# Autodesk Inventor assembly: GE-12089
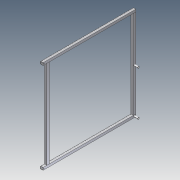
[picture p0: Inventor's stored thumbnail of the model, 180x180]
Saved by Autodesk Inventor 2012 (Build 160160000, 160)
## iProperties
Created: 2011-10-10
Part Number: GE-12089
Document SubType Name: Assembly
Designer: dfoster
Description: Corral Frame, Right
Title: Corral Frame, Right
Author: dfoster
## Documents named in this file (4)
- C:\Data Folder\FRC 2012 Field\Components\GE-12089.iam
- C:\Data Folder\FRC 2012 Field\Components\GE-12089-01.ipt
- C:\Data Folder\FRC 2012 Field\Components\GE-12089-02.ipt
- C:\Data Folder\FRC 2012 Field\Components\GE-12089-03.ipt
## Components (6 placed, 3 different names)
1. GE-12089-01:1 — Flush:1, Mate:1, Flush:2, Flush:3, Flush:5, Flush:6
2. GE-12089-01:2 — Mate:2, Flush:4, Flush:5
3. GE-12089-02:1 — Flush:1
4. GE-12089-02:2 — Mate:1, Flush:2, Flush:3, Mate:2, Flush:4
5. GE-12089-03:1 — Flush:6
6. GE-12089-03:2
## Relationships (13: Mate 7, Flush 6)
- Flush:1: GE-12089-01:1 ↔ GE-12089-02:1
- Mate:1: GE-12089-01:1 ↔ GE-12089-02:2
- Flush:2: GE-12089-01:1 ↔ GE-12089-02:2
- Flush:3 (50.8 mm): GE-12089-01:1 ↔ GE-12089-02:2
- Mate:2: GE-12089-01:2 ↔ GE-12089-02:2
- Flush:4: GE-12089-01:2 ↔ GE-12089-02:2
- Flush:5: GE-12089-01:1 ↔ GE-12089-01:2
- Flush:6: GE-12089-01:1 ↔ GE-12089-03:1
- [Mate] (-15.875 mm): GE-12089-01:1 ↔ GE-12089-03:1
- [Mate] (-15.875 mm): GE-12089-01:1 ↔ GE-12089-03:1
- [Mate]: GE-12089-02:1 ↔ GE-12089-03:2
- [Mate] (-15.875 mm): GE-12089-02:1 ↔ GE-12089-03:2
- [Mate] (-593.725 mm): GE-12089-01:1 ↔ GE-12089-03:2
